# Autodesk Inventor assembly: stepperMotorBodyPlusAxel
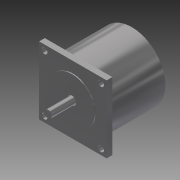
[picture p0: Inventor's stored thumbnail of the model, 180x180]
Saved by Autodesk Inventor 2013 (Build 170138000, 138)
## iProperties
Created: 2013-02-25
Part Number: stepperMotorBodyPlusAxel
Document SubType Name: Assembly
Designer: Nano
Author: Nano
## Documents named in this file (3)
- C:\Users\Nano\Documents\InventorByron\InventorMasterProject\gyroPhone01\stepperMotorBodyPlusAxel.iam
- C:\Users\Nano\Documents\InventorByron\InventorMasterProject\gyroPhone01\stepperMotorBody.ipt
- C:\Users\Nano\Documents\InventorByron\InventorMasterProject\gyroPhone01\stepperMotorAxel.ipt
## Components (2 placed, 2 different names)
1. stepperMotorBody:1 — Mate:1, Flush:1
2. stepperMotorAxel:1 — Mate:1, Flush:1
## Relationships (2: Mate 1, Flush 1)
- Mate:1: stepperMotorBody:1 ↔ stepperMotorAxel:1
- Flush:1: stepperMotorBody:1 ↔ stepperMotorAxel:1
